# Autodesk Inventor assembly: dial-indicator-holder-assembly
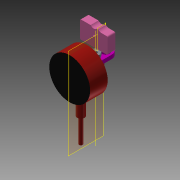
[picture p0: Inventor's stored thumbnail of the model, 180x180]
Saved by Autodesk Inventor 2014 (Build 180170000, 170)
## iProperties
Created: 2013-12-31
Part Number: dial-indicator-holder-assembly
Document SubType Name: Assembly
Designer: caleb
Author: caleb
## Documents named in this file (7)
- C:\cygwin\home\caleb\caleb-typea-settings\designs\dial-gauge-holder\dial-indicator-holder-assembly.iam
- C:\cygwin\home\caleb\caleb-typea-settings\designs\dial-gauge-holder\dial-indicator.ipt
- C:\cygwin\home\caleb\caleb-typea-settings\designs\dial-gauge-holder\hotend-holder-front.ipt
- C:\cygwin\home\caleb\caleb-typea-settings\designs\dial-gauge-holder\peek-insulator.ipt
- C:\cygwin\home\caleb\caleb-typea-settings\designs\dial-gauge-holder\dial-indicator-holder.ipt
- C:\Documents and Settings\caleb\My Documents\Inventor\Content Center Files\R2014\en-US\ANSI B18.2.2(09)\ANSI B18.2.2 - 1_4 - 20(2).ipt
- C:\Documents and Settings\caleb\My Documents\Inventor\Content Center Files\R2014\en-US\ANSI ASME B18.2.1(2)\ANSI_ASME B18.2.1 - 1_4-20 UNC - 0.5(2).ipt
## Components (6 placed, 6 different names)
1. dial-indicator:1 — Flush:1, Mate:7, Mate:12, Mate:13
2. hotend-holder-front:1 — Mate:1, Mate:2, Mate:3, Mate:4, Flush:1, Mate:5, Mate:8
3. peek-insulator:1 — Mate:3, Mate:4
4. dial-indicator-holder:1 — Mate:5, Mate:7, Mate:8, Mate:9, Mate:10
5. Hex Nut - Inch 1/4 - 20:1 — Mate:9, Mate:10, Mate:11
6. Hex Bolt - Inch 1/4-20 UNC - 0.5:1 — Mate:11, Mate:12, Mate:13
## Relationships (13: Mate 12, Flush 1)
- Mate:1: hotend-holder-front:1
- Mate:2: hotend-holder-front:1
- Mate:3: hotend-holder-front:1 ↔ peek-insulator:1
- Mate:4: hotend-holder-front:1 ↔ peek-insulator:1
- Flush:1: dial-indicator:1 ↔ hotend-holder-front:1
- Mate:5: hotend-holder-front:1 ↔ dial-indicator-holder:1
- Mate:7: dial-indicator:1 ↔ dial-indicator-holder:1
- Mate:8: hotend-holder-front:1 ↔ dial-indicator-holder:1
- Mate:9: dial-indicator-holder:1 ↔ Hex Nut - Inch 1/4 - 20:1
- Mate:10: dial-indicator-holder:1 ↔ Hex Nut - Inch 1/4 - 20:1
- Mate:11: Hex Nut - Inch 1/4 - 20:1 ↔ Hex Bolt - Inch 1/4-20 UNC - 0.5:1
- Mate:12: dial-indicator:1 ↔ Hex Bolt - Inch 1/4-20 UNC - 0.5:1
- Mate:13: dial-indicator:1 ↔ Hex Bolt - Inch 1/4-20 UNC - 0.5:1
